# Autodesk Inventor assembly: mountAssembly
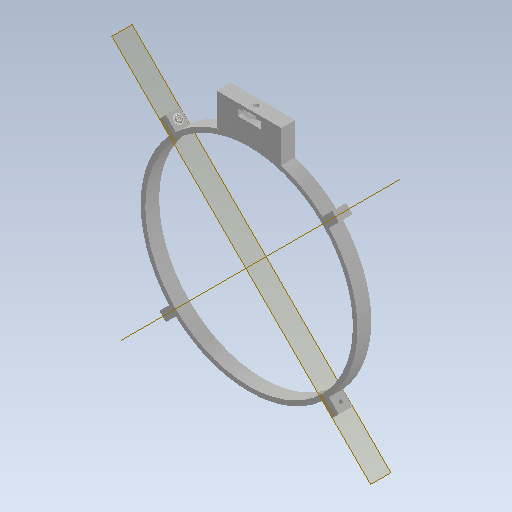
[picture p0: Inventor's stored thumbnail of the model, 512x512]
Saved by Autodesk Inventor 2021 (Build 250183000, 183)
## iProperties
Created: 2020-07-16
Part Number: mountAssembly
Document SubType Name: Assembly
Designer: robst
Author: robst
## Documents named in this file (6)
- C:\git\CAD-Development\robSteele\ShapeWays\TelescopeProjects\cameraMountForLx200\mountAssembly.iam
- C:\git\CAD-Development\robSteele\ShapeWays\TelescopeProjects\cameraMountForLx200\mount.ipt
- C:\Users\robst\Documents\Inventor\Content Center Files\R2021\en-US\ANSI B18.22.1\ANSI B18.22.1 - No. 10 - Type A.ipt
- C:\Users\robst\Documents\Inventor\Content Center Files\R2021\en-US\U UNC 2605\Unbrako - 10 x 3_4 - 32(10).ipt
- C:\Users\robst\Documents\Inventor\Content Center Files\R2021\en-US\ANSI B 18.2.2(2)\ANSI B 18.2.2 - #10-32(2).ipt
- C:\git\CAD-Development\robSteele\ShapeWays\TelescopeProjects\cameraMountForLx200\knurledKnob.ipt
## Components (6 placed, 5 different names)
1. mount:1 — Mate:3, Mate:4, Mate:5, Mate:6, Insert:4
2. Plain Washer (Inch) No. 10 - Type A:1 — Mate:3, Mate:4, Insert:2
3. Unbrako UNC Hex Socket Button Cap - Inch 10 x 3/4:1 — Insert:2
4. Plain Washer (Inch) No. 10 - Type A:2 — Mate:5, Mate:6, Insert:3
5. Low Crown #10-32:1 — Insert:3
6. knurledKnob:1 — Insert:4
## Relationships (7: Mate 4, Insert 3)
- Mate:3: mount:1 ↔ Plain Washer (Inch) No. 10 - Type A:1
- Mate:4: mount:1 ↔ Plain Washer (Inch) No. 10 - Type A:1
- Insert:2: Plain Washer (Inch) No. 10 - Type A:1 ↔ Unbrako UNC Hex Socket Button Cap - Inch 10 x 3/4:1
- Mate:5: mount:1 ↔ Plain Washer (Inch) No. 10 - Type A:2
- Mate:6: mount:1 ↔ Plain Washer (Inch) No. 10 - Type A:2
- Insert:3: Plain Washer (Inch) No. 10 - Type A:2 ↔ Low Crown #10-32:1
- Insert:4: mount:1 ↔ knurledKnob:1
